# Autodesk Inventor assembly: VolteraOne_tool.ipj
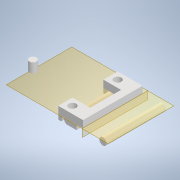
[picture p0: Inventor's stored thumbnail of the model, 180x180]
Saved by Autodesk Inventor 2022 (Build 260153000, 153)
## iProperties
Created: 2022-08-22
Part Number: VolteraOne_tool.ipj
Document SubType Name: Assembly
Designer: diederichbenedict
Author: diederichbenedict
## Documents named in this file (4)
- C:\Users\diederichbenedict\Dropbox\Dokumente\Promotion\PROJECTS\VOLTERA\INVENTOR\VolteraOne_tool.ipj.iam
- C:\Users\diederichbenedict\Dropbox\Dokumente\Promotion\PROJECTS\VOLTERA\INVENTOR\00_rod_6mm.ipt
- C:\Users\diederichbenedict\Dropbox\Dokumente\Promotion\PROJECTS\VOLTERA\INVENTOR\00_Magnets_6x8mm.ipt
- C:\Users\diederichbenedict\Dropbox\Dokumente\Promotion\PROJECTS\VOLTERA\INVENTOR\Voltera_Slide.ipt
## Components (4 placed, 3 different names)
1. 00_Magnets_6x8mm:1
2. Voltera_Slide:1 — Fluchtend:2, Fluchtend:3
3. 00_rod_6mm:1 — Symmetrie:1
4. 00_rod_6mm:2 — Symmetrie:1
## Component patterns: (2 elements, first: 00_rod_6mm:1)
## Relationships (4: Flush 3, Symmetry 1)
- Fluchtend:1 [Flush] (3 mm)
- Symmetrie:1: 00_rod_6mm:1 ↔ 00_rod_6mm:2
- Fluchtend:2 [Flush]: Voltera_Slide:1
- Fluchtend:3 [Flush]: Voltera_Slide:1
